# Autodesk Inventor assembly: Sheep
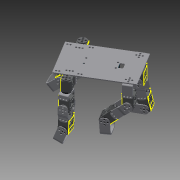
[picture p0: Inventor's stored thumbnail of the model, 180x180]
Saved by Autodesk Inventor 2014 SP1 (Build 180222100, 222)
## iProperties
Created: 2014-04-23
Part Number: Sheep
Document SubType Name: Assembly
Designer: david
Author: david
## Documents named in this file (11)
- C:\Users\asus\Documents\GitHub\SheepWarrior\Autodesk\V2\Sheep\Sheep.iam
- C:\Users\asus\Documents\GitHub\SheepWarrior\Autodesk\V2\Sheep\Body.ipt
- C:\Users\asus\Documents\GitHub\SheepWarrior\Autodesk\V2\Sheep\Equerre.ipt
- C:\Users\asus\Documents\GitHub\SheepWarrior\Autodesk\V2\XL320\src\Motor.iam
- C:\Users\asus\Documents\GitHub\SheepWarrior\Autodesk\V2\XL320\src\Pantilt.ipt
- C:\Users\asus\Documents\GitHub\SheepWarrior\Autodesk\V2\XL320\src\ArmToBottom.ipt
- C:\Users\asus\Documents\GitHub\SheepWarrior\Autodesk\V2\Sheep\Board.ipt
- C:\Users\asus\Documents\GitHub\SheepWarrior\Autodesk\V2\Sheep\BackLegUpperBone.ipt
- C:\Users\asus\Documents\GitHub\SheepWarrior\Autodesk\V2\Sheep\BackLegMiddleBone.ipt
- C:\Users\asus\Documents\GitHub\SheepWarrior\Autodesk\V2\Sheep\BackFeet.ipt
- C:\Users\asus\Documents\GitHub\SheepWarrior\Autodesk\V2\Sheep\FrontFeet.ipt
## Components (32 placed, 10 different names)
1. Body:1 — Mate:8, Mate:9, Mate:11, Mate:12, Mate:14, Mate:15, Mate:16, Mate:54, Mate:55, Mate:56, Mate:57, Mate:58, Mate:59, Mate:60, Mate:61, Mate:62, Mate:73, Angle:1, Mate:74, Mate:75, Mate:76, Mate:77, Mate:78, Mate:82, Mate:83, Mate:84
2. Equerre:1 — Mate:8, Mate:9
3. Equerre:2 — Mate:11, Mate:12
4. Motor:1 [sub-assembly] — Mate:14, Mate:15, Mate:16, Mate:17, Rotational:1
5. Pantilt:1 — Mate:17, Rotational:1, Mate:18, Mate:19, Mate:20
6. Motor:2 [sub-assembly] — Mate:18, Mate:19, Mate:20, Mate:21, Mate:24, Rotational:2, Rotational:3
7. ArmToBottom:1 — Mate:21, Rotational:3, Mate:25, Mate:26, Mate:27
8. ArmToBottom:2 — Mate:24, Rotational:2, Mate:28
9. Motor:3 [sub-assembly] — Mate:25, Mate:26, Mate:27, Mate:28, Mate:102, Rotational:20
10. Motor:4 [sub-assembly] — Mate:85, Mate:86, Mate:87, Mate:91, Mate:92, Mate:93, Rotational:17
11. Motor:5 [sub-assembly] — Mate:94, Mate:95, Mate:97, Mate:99, Mate:100
12. Motor:6 [sub-assembly] — Mate:79, Mate:80, Mate:81, Mate:88, Rotational:15, Rotational:16
13. Motor:7 [sub-assembly] — Mate:89, Mate:90, Mate:96, Mate:98, Rotational:18
14. Equerre:3 — Mate:54, Mate:58, Mate:59
15. Equerre:4 — Mate:55, Mate:56, Mate:57
16. Motor:8 [sub-assembly] — Mate:60, Mate:61, Mate:62, Mate:63, Rotational:11
17. Motor:9 [sub-assembly] — Mate:69, Mate:70, Mate:71, Mate:101, Rotational:19
18. Motor:10 [sub-assembly] — Mate:64, Mate:65, Mate:66, Mate:67, Rotational:12, Mate:68, Rotational:13
19. Pantilt:4 — Mate:63, Rotational:11, Mate:64, Mate:65, Mate:66
20. ArmToBottom:7 — Mate:67, Rotational:12, Mate:69, Mate:70
21. ArmToBottom:8 — Mate:68, Rotational:13, Mate:71
22. Board:1 — Mate:73, Angle:1, Mate:74
23. BackLegUpperBone:1 — Mate:75, Mate:76, Mate:77, Mate:78, Mate:79, Mate:80, Mate:81
24. BackLegUpperBone:2 — Mate:82, Mate:83, Mate:84, Mate:85, Mate:86, Mate:87
25. BackLegMiddleBone:1 — Rotational:16, Mate:90
26. BackLegMiddleBone:2 — Mate:88, Rotational:15, Mate:89, Mate:96
27. BackLegMiddleBone:3 — Mate:91, Mate:92, Mate:95
28. BackLegMiddleBone:4 — Mate:93, Rotational:17, Mate:94, Mate:97
29. BackFeet:1 — Mate:98, Rotational:18
30. BackFeet:2 — Mate:99, Mate:100
31. FrontFeet:1 — Mate:101, Rotational:19
32. FrontFeet:2 — Mate:102, Rotational:20
## Relationships (78: Mate 65, RevoluteJoint 12, Angle 1)
- Mate:8: Body:1 ↔ Equerre:1
- Mate:9: Body:1 ↔ Equerre:1
- Mate:11: Body:1 ↔ Equerre:2
- Mate:12: Body:1 ↔ Equerre:2
- Mate:14: Body:1 ↔ Motor:1
- Mate:15: Body:1 ↔ Motor:1
- Mate:16: Body:1 ↔ Motor:1
- Mate:17: Motor:1 ↔ Pantilt:1
- Rotational:1 [RevoluteJoint]: Motor:1 ↔ Pantilt:1
- Mate:18: Pantilt:1 ↔ Motor:2
- Mate:19: Pantilt:1 ↔ Motor:2
- Mate:20: Pantilt:1 ↔ Motor:2
- Mate:21: Motor:2 ↔ ArmToBottom:1
- Mate:24: Motor:2 ↔ ArmToBottom:2
- Rotational:2 [RevoluteJoint]: Motor:2 ↔ ArmToBottom:2
- Rotational:3 [RevoluteJoint]: Motor:2 ↔ ArmToBottom:1
- Mate:25: ArmToBottom:1 ↔ Motor:3
- Mate:26: ArmToBottom:1 ↔ Motor:3
- Mate:27: ArmToBottom:1 ↔ Motor:3
- Mate:28: ArmToBottom:2 ↔ Motor:3
- Mate:54: Body:1 ↔ Equerre:3
- Mate:55: Body:1 ↔ Equerre:4
- Mate:56: Body:1 ↔ Equerre:4
- Mate:57: Body:1 ↔ Equerre:4
- Mate:58: Body:1 ↔ Equerre:3
- Mate:59: Body:1 ↔ Equerre:3
- Mate:60: Body:1 ↔ Motor:8
- Mate:61: Body:1 ↔ Motor:8
- Mate:62: Body:1 ↔ Motor:8
- Mate:63: Motor:8 ↔ Pantilt:4
- Rotational:11 [RevoluteJoint]: Motor:8 ↔ Pantilt:4
- Mate:64: Motor:10 ↔ Pantilt:4
- Mate:65: Motor:10 ↔ Pantilt:4
- Mate:66: Motor:10 ↔ Pantilt:4
- Mate:67: Motor:10 ↔ ArmToBottom:7
- Rotational:12 [RevoluteJoint]: Motor:10 ↔ ArmToBottom:7
- Mate:68: Motor:10 ↔ ArmToBottom:8
- Rotational:13 [RevoluteJoint]: Motor:10 ↔ ArmToBottom:8
- Mate:69: Motor:9 ↔ ArmToBottom:7
- Mate:70: Motor:9 ↔ ArmToBottom:7
- Mate:71: Motor:9 ↔ ArmToBottom:8
- Mate:73: Body:1 ↔ Board:1
- Angle:1 (0 deg): Body:1 ↔ Board:1
- Mate:74: Body:1 ↔ Board:1
- Mate:75: Body:1 ↔ BackLegUpperBone:1
- Mate:76: Body:1 ↔ BackLegUpperBone:1
- Mate:77: Body:1 ↔ BackLegUpperBone:1
- Mate:78: Body:1 ↔ BackLegUpperBone:1
- Mate:79: Motor:6 ↔ BackLegUpperBone:1
- Mate:80: Motor:6 ↔ BackLegUpperBone:1
- Mate:81: Motor:6 ↔ BackLegUpperBone:1
- Mate:82: Body:1 ↔ BackLegUpperBone:2
- Mate:83: Body:1 ↔ BackLegUpperBone:2
- Mate:84: Body:1 ↔ BackLegUpperBone:2
- Mate:85: Motor:4 ↔ BackLegUpperBone:2
- Mate:86: Motor:4 ↔ BackLegUpperBone:2
- Mate:87: Motor:4 ↔ BackLegUpperBone:2
- Mate:88: Motor:6 ↔ BackLegMiddleBone:2
- Rotational:15 [RevoluteJoint]: Motor:6 ↔ BackLegMiddleBone:2
- Rotational:16 [RevoluteJoint]: Motor:6 ↔ BackLegMiddleBone:1
- Mate:89: Motor:7 ↔ BackLegMiddleBone:2
- Mate:90: Motor:7 ↔ BackLegMiddleBone:1
- Mate:91: Motor:4 ↔ BackLegMiddleBone:3
- Mate:92: Motor:4 ↔ BackLegMiddleBone:3
- Mate:93: Motor:4 ↔ BackLegMiddleBone:4
- Rotational:17 [RevoluteJoint]: Motor:4 ↔ BackLegMiddleBone:4
- Mate:94: Motor:5 ↔ BackLegMiddleBone:4
- Mate:95: Motor:5 ↔ BackLegMiddleBone:3
- Mate:96: Motor:7 ↔ BackLegMiddleBone:2
- Mate:97: Motor:5 ↔ BackLegMiddleBone:4
- Mate:98: Motor:7 ↔ BackFeet:1
- Rotational:18 [RevoluteJoint]: Motor:7 ↔ BackFeet:1
- Mate:99: Motor:5 ↔ BackFeet:2
- Mate:100: Motor:5 ↔ BackFeet:2
- Mate:101: Motor:9 ↔ FrontFeet:1
- Mate:102: Motor:3 ↔ FrontFeet:2
- Rotational:19 [RevoluteJoint]: Motor:9 ↔ FrontFeet:1
- Rotational:20 [RevoluteJoint]: Motor:3 ↔ FrontFeet:2
